# Autodesk Inventor assembly: leg_Left_femur_ass
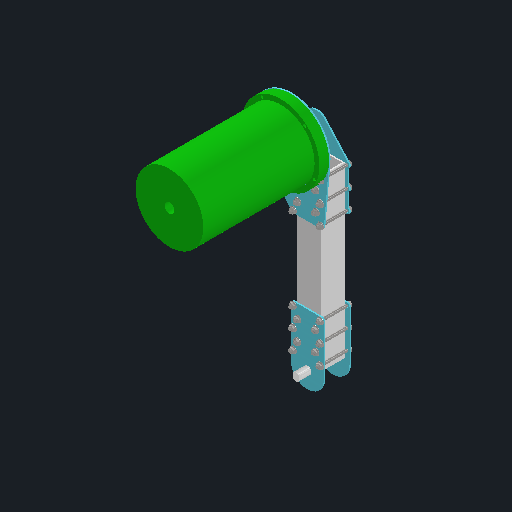
[picture p0: Inventor's stored thumbnail of the model, 512x512]
Saved by Autodesk Inventor 2026 (Build 300175000, 175)
## iProperties
Created: 2026-04-24
Part Number: leg_Left_femur_ass
Document SubType Name: Assembly
Designer: user
Mass: 1158.5 g
Surface Area: 2231.02 cm^2
Volume: 319.422 cm^3
Author: user
## Documents named in this file (10)
- C:\Users\user\vs_code_projects\ogonek-spider\physical-structure\cad\leg_femur\leg_Right_femur_ass.iam
- C:\Users\user\vs_code_projects\ogonek-spider\physical-structure\cad\leg_femur\femur_profile.ipt
- C:\Users\user\vs_code_projects\ogonek-spider\physical-structure\cad\leg_femur\femur_support_steel.ipt
- C:\Users\user\vs_code_projects\ogonek-spider\physical-structure\cad\leg_femur\femur_motor_steel.ipt
- C:\Users\user\vs_code_projects\ogonek-spider\physical-structure\cad\leg_femur\femur_outside_steel.ipt
- C:\Users\user\Documents\Inventor\Content Center Files\R2026\ru-RU\GOST 7805-70\Болт M6-6gx65 ГОСТ 7805-70.ipt
- C:\Users\user\Documents\Inventor\Content Center Files\R2026\ru-RU\Nut GOST R 50592-93\Гайка M6-6H ГОСТ Р 50592-93.ipt
- C:\Users\user\Documents\Inventor\Content Center Files\R2026\ru-RU\GOST 7798-70\Болт M6-6gx65 ГОСТ 7798-70.ipt
- C:\Users\user\vs_code_projects\ogonek-spider\physical-structure\cad\leg_femur\shaft_femur.ipt
- C:\Users\user\vs_code_projects\ogonek-spider\physical-structure\cad\body_parts\motor_mass.ipt
## Components (47 placed, 9 different names)
1. femur_profile:1 — Жесткий:2, Жесткий:3, Совмещение:47, Совмещение:67, С поворотом:1, С поворотом:2, С поворотом:3, С поворотом:4
2. femur_support_steel:1 — Жесткий:6, Жесткий:7, Жесткий:8, Жесткий:9, Жесткий:10, Жесткий:11, Жесткий:12, Жесткий:13, Жесткий:14, Жесткий:15, С поворотом:1, С поворотом:2
3. femur_motor_steel:1 — С поворотом:3, С поворотом:4, С поворотом:5, С поворотом:6, С поворотом:7, С поворотом:8, С поворотом:9, С поворотом:10, С поворотом:11, С поворотом:12, С поворотом:13, С поворотом:14, С поворотом:15, С поворотом:16
4. femur_outside_steel:1 — Жесткий:2, Совмещение:62, Совмещение:64, Совмещение:66, Совмещение:68, Совмещение:70, Совмещение:72, Совмещение:74, Совмещение:76, Совмещение:78, Совмещение:80
5. femur_outside_steel:2 — Жесткий:3, Совмещение:41, Совмещение:42, Совмещение:43, Совмещение:44, Совмещение:45, Совмещение:46, Совмещение:48, Совмещение:49, Совмещение:50, Совмещение:51, Совмещение:52, Совмещение:53, Совмещение:54, Совмещение:55, Совмещение:56, Совмещение:57, Совмещение:58, Совмещение:59, Совмещение:60, Совмещение:61, Совмещение:63, Совмещение:65, Совмещение:69, Совмещение:71, Совмещение:73, Совмещение:75, Совмещение:77, Совмещение:79, Жесткий:5
6. shaft_femur:1 — Жесткий:5
7. motor_mass:1 — С поворотом:15, С поворотом:16
8. Болт ГОСТ 7798-70 - Отозвано M6-6gx65:1 — Совмещение:41, Совмещение:42
9. Гайка ГОСТ Р 50592-93 M6:11 — Совмещение:61, Совмещение:62
10. Болт ГОСТ 7798-70 - Отозвано M6-6gx65:2 — Совмещение:43, Совмещение:44
11. Болт ГОСТ 7798-70 - Отозвано M6-6gx65:3 — Совмещение:45, Совмещение:46
12. Болт ГОСТ 7798-70 - Отозвано M6-6gx65:4 — Совмещение:47, Совмещение:48
13. Болт ГОСТ 7798-70 - Отозвано M6-6gx65:5 — Совмещение:49, Совмещение:50
14. Болт ГОСТ 7798-70 - Отозвано M6-6gx65:6 — Совмещение:51, Совмещение:52
15. Болт ГОСТ 7798-70 - Отозвано M6-6gx65:7 — Совмещение:53, Совмещение:54
16. Болт ГОСТ 7798-70 - Отозвано M6-6gx65:8 — Совмещение:55, Совмещение:56
17. Болт ГОСТ 7798-70 - Отозвано M6-6gx65:9 — Совмещение:57, Совмещение:58
18. Болт ГОСТ 7798-70 - Отозвано M6-6gx65:10 — Совмещение:59, Совмещение:60
19. Гайка ГОСТ Р 50592-93 M6:12 — Совмещение:63, Совмещение:64
20. Гайка ГОСТ Р 50592-93 M6:13 — Совмещение:65, Совмещение:66
21. Гайка ГОСТ Р 50592-93 M6:14 — Совмещение:67, Совмещение:68
22. Гайка ГОСТ Р 50592-93 M6:15 — Совмещение:69, Совмещение:70
23. Гайка ГОСТ Р 50592-93 M6:16 — Совмещение:71, Совмещение:72
24. Гайка ГОСТ Р 50592-93 M6:17 — Совмещение:73, Совмещение:74
25. Гайка ГОСТ Р 50592-93 M6:18 — Совмещение:75, Совмещение:76
26. Гайка ГОСТ Р 50592-93 M6:19 — Совмещение:77, Совмещение:78
27. Гайка ГОСТ Р 50592-93 M6:20 — Совмещение:79, Совмещение:80
28. Болт ГОСТ 7805-70 M6-6gx65:1 — Жесткий:9
29. Гайка ГОСТ Р 50592-93 M6:1 — С поворотом:5
30. Болт ГОСТ 7805-70 M6-6gx65:2 — Жесткий:8
31. Болт ГОСТ 7805-70 M6-6gx65:3 — Жесткий:6
32. Болт ГОСТ 7805-70 M6-6gx65:4 — Жесткий:10
33. Болт ГОСТ 7805-70 M6-6gx65:5 — Жесткий:7
34. Болт ГОСТ 7805-70 M6-6gx65:6 — Жесткий:11
35. Болт ГОСТ 7805-70 M6-6gx65:7 — Жесткий:12
36. Болт ГОСТ 7805-70 M6-6gx65:8 — Жесткий:13
37. Болт ГОСТ 7805-70 M6-6gx65:9 — Жесткий:15
38. Болт ГОСТ 7805-70 M6-6gx65:10 — Жесткий:14
39. Гайка ГОСТ Р 50592-93 M6:2 — С поворотом:7
40. Гайка ГОСТ Р 50592-93 M6:3 — С поворотом:14
41. Гайка ГОСТ Р 50592-93 M6:4 — С поворотом:8
42. Гайка ГОСТ Р 50592-93 M6:5 — С поворотом:12
43. Гайка ГОСТ Р 50592-93 M6:6 — С поворотом:11
44. Гайка ГОСТ Р 50592-93 M6:7 — С поворотом:13
45. Гайка ГОСТ Р 50592-93 M6:8 — С поворотом:6
46. Гайка ГОСТ Р 50592-93 M6:9 — С поворотом:10
47. Гайка ГОСТ Р 50592-93 M6:10 — С поворотом:9
## Relationships (69: Mate 40, RevoluteJoint 16, WeldJoint 13)
- Жесткий:2 [WeldJoint]: femur_profile:1 ↔ femur_outside_steel:1
- Жесткий:3 [WeldJoint]: femur_profile:1 ↔ femur_outside_steel:2
- Совмещение:41 [Mate]: femur_outside_steel:2 ↔ Болт ГОСТ 7798-70 - Отозвано M6-6gx65:1
- Совмещение:42 [Mate]: femur_outside_steel:2 ↔ Болт ГОСТ 7798-70 - Отозвано M6-6gx65:1
- Совмещение:43 [Mate]: femur_outside_steel:2 ↔ Болт ГОСТ 7798-70 - Отозвано M6-6gx65:2
- Совмещение:44 [Mate]: femur_outside_steel:2 ↔ Болт ГОСТ 7798-70 - Отозвано M6-6gx65:2
- Совмещение:45 [Mate]: femur_outside_steel:2 ↔ Болт ГОСТ 7798-70 - Отозвано M6-6gx65:3
- Совмещение:46 [Mate]: femur_outside_steel:2 ↔ Болт ГОСТ 7798-70 - Отозвано M6-6gx65:3
- Совмещение:47 [Mate]: femur_profile:1 ↔ Болт ГОСТ 7798-70 - Отозвано M6-6gx65:4
- Совмещение:48 [Mate]: femur_outside_steel:2 ↔ Болт ГОСТ 7798-70 - Отозвано M6-6gx65:4
- Совмещение:49 [Mate]: femur_outside_steel:2 ↔ Болт ГОСТ 7798-70 - Отозвано M6-6gx65:5
- Совмещение:50 [Mate]: femur_outside_steel:2 ↔ Болт ГОСТ 7798-70 - Отозвано M6-6gx65:5
- Совмещение:51 [Mate]: femur_outside_steel:2 ↔ Болт ГОСТ 7798-70 - Отозвано M6-6gx65:6
- Совмещение:52 [Mate]: femur_outside_steel:2 ↔ Болт ГОСТ 7798-70 - Отозвано M6-6gx65:6
- Совмещение:53 [Mate]: femur_outside_steel:2 ↔ Болт ГОСТ 7798-70 - Отозвано M6-6gx65:7
- Совмещение:54 [Mate]: femur_outside_steel:2 ↔ Болт ГОСТ 7798-70 - Отозвано M6-6gx65:7
- Совмещение:55 [Mate]: femur_outside_steel:2 ↔ Болт ГОСТ 7798-70 - Отозвано M6-6gx65:8
- Совмещение:56 [Mate]: femur_outside_steel:2 ↔ Болт ГОСТ 7798-70 - Отозвано M6-6gx65:8
- Совмещение:57 [Mate]: femur_outside_steel:2 ↔ Болт ГОСТ 7798-70 - Отозвано M6-6gx65:9
- Совмещение:58 [Mate]: femur_outside_steel:2 ↔ Болт ГОСТ 7798-70 - Отозвано M6-6gx65:9
- Совмещение:59 [Mate]: femur_outside_steel:2 ↔ Болт ГОСТ 7798-70 - Отозвано M6-6gx65:10
- Совмещение:60 [Mate]: femur_outside_steel:2 ↔ Болт ГОСТ 7798-70 - Отозвано M6-6gx65:10
- Совмещение:61 [Mate]: femur_outside_steel:2 ↔ Гайка ГОСТ Р 50592-93 M6:11
- Совмещение:62 [Mate]: femur_outside_steel:1 ↔ Гайка ГОСТ Р 50592-93 M6:11
- Совмещение:63 [Mate]: femur_outside_steel:2 ↔ Гайка ГОСТ Р 50592-93 M6:12
- Совмещение:64 [Mate]: femur_outside_steel:1 ↔ Гайка ГОСТ Р 50592-93 M6:12
- Совмещение:65 [Mate]: femur_outside_steel:2 ↔ Гайка ГОСТ Р 50592-93 M6:13
- Совмещение:66 [Mate]: femur_outside_steel:1 ↔ Гайка ГОСТ Р 50592-93 M6:13
- Совмещение:67 [Mate]: femur_profile:1 ↔ Гайка ГОСТ Р 50592-93 M6:14
- Совмещение:68 [Mate]: femur_outside_steel:1 ↔ Гайка ГОСТ Р 50592-93 M6:14
- Совмещение:69 [Mate]: femur_outside_steel:2 ↔ Гайка ГОСТ Р 50592-93 M6:15
- Совмещение:70 [Mate]: femur_outside_steel:1 ↔ Гайка ГОСТ Р 50592-93 M6:15
- Совмещение:71 [Mate]: femur_outside_steel:2 ↔ Гайка ГОСТ Р 50592-93 M6:16
- Совмещение:72 [Mate]: femur_outside_steel:1 ↔ Гайка ГОСТ Р 50592-93 M6:16
- Совмещение:73 [Mate]: femur_outside_steel:2 ↔ Гайка ГОСТ Р 50592-93 M6:17
- Совмещение:74 [Mate]: femur_outside_steel:1 ↔ Гайка ГОСТ Р 50592-93 M6:17
- Совмещение:75 [Mate]: femur_outside_steel:2 ↔ Гайка ГОСТ Р 50592-93 M6:18
- Совмещение:76 [Mate]: femur_outside_steel:1 ↔ Гайка ГОСТ Р 50592-93 M6:18
- Совмещение:77 [Mate]: femur_outside_steel:2 ↔ Гайка ГОСТ Р 50592-93 M6:19
- Совмещение:78 [Mate]: femur_outside_steel:1 ↔ Гайка ГОСТ Р 50592-93 M6:19
- Совмещение:79 [Mate]: femur_outside_steel:2 ↔ Гайка ГОСТ Р 50592-93 M6:20
- Совмещение:80 [Mate]: femur_outside_steel:1 ↔ Гайка ГОСТ Р 50592-93 M6:20
- Жесткий:5 [WeldJoint] (20 mm): femur_outside_steel:2 ↔ shaft_femur:1
- Жесткий:6 [WeldJoint]: femur_support_steel:1 ↔ Болт ГОСТ 7805-70 M6-6gx65:3
- Жесткий:7 [WeldJoint]: femur_support_steel:1 ↔ Болт ГОСТ 7805-70 M6-6gx65:5
- Жесткий:8 [WeldJoint]: femur_support_steel:1 ↔ Болт ГОСТ 7805-70 M6-6gx65:2
- Жесткий:9 [WeldJoint]: femur_support_steel:1 ↔ Болт ГОСТ 7805-70 M6-6gx65:1
- Жесткий:10 [WeldJoint]: femur_support_steel:1 ↔ Болт ГОСТ 7805-70 M6-6gx65:4
- Жесткий:11 [WeldJoint]: femur_support_steel:1 ↔ Болт ГОСТ 7805-70 M6-6gx65:6
- Жесткий:12 [WeldJoint]: femur_support_steel:1 ↔ Болт ГОСТ 7805-70 M6-6gx65:7
- Жесткий:13 [WeldJoint]: femur_support_steel:1 ↔ Болт ГОСТ 7805-70 M6-6gx65:8
- Жесткий:14 [WeldJoint]: femur_support_steel:1 ↔ Болт ГОСТ 7805-70 M6-6gx65:10
- Жесткий:15 [WeldJoint]: femur_support_steel:1 ↔ Болт ГОСТ 7805-70 M6-6gx65:9
- С поворотом:1 [RevoluteJoint]: femur_profile:1 ↔ femur_support_steel:1
- С поворотом:2 [RevoluteJoint]: femur_profile:1 ↔ femur_support_steel:1
- С поворотом:3 [RevoluteJoint]: femur_profile:1 ↔ femur_motor_steel:1
- С поворотом:4 [RevoluteJoint]: femur_profile:1 ↔ femur_motor_steel:1
- С поворотом:5 [RevoluteJoint]: femur_motor_steel:1 ↔ Гайка ГОСТ Р 50592-93 M6:1
- С поворотом:6 [RevoluteJoint]: femur_motor_steel:1 ↔ Гайка ГОСТ Р 50592-93 M6:8
- С поворотом:7 [RevoluteJoint]: femur_motor_steel:1 ↔ Гайка ГОСТ Р 50592-93 M6:2
- С поворотом:8 [RevoluteJoint]: femur_motor_steel:1 ↔ Гайка ГОСТ Р 50592-93 M6:4
- С поворотом:9 [RevoluteJoint]: femur_motor_steel:1 ↔ Гайка ГОСТ Р 50592-93 M6:10
- С поворотом:10 [RevoluteJoint]: femur_motor_steel:1 ↔ Гайка ГОСТ Р 50592-93 M6:9
- С поворотом:11 [RevoluteJoint]: femur_motor_steel:1 ↔ Гайка ГОСТ Р 50592-93 M6:6
- С поворотом:12 [RevoluteJoint]: femur_motor_steel:1 ↔ Гайка ГОСТ Р 50592-93 M6:5
- С поворотом:13 [RevoluteJoint]: femur_motor_steel:1 ↔ Гайка ГОСТ Р 50592-93 M6:7
- С поворотом:14 [RevoluteJoint]: femur_motor_steel:1 ↔ Гайка ГОСТ Р 50592-93 M6:3
- С поворотом:15 [RevoluteJoint]: femur_motor_steel:1 ↔ motor_mass:1
- С поворотом:16 [RevoluteJoint]: femur_motor_steel:1 ↔ motor_mass:1
